# Autodesk Inventor assembly: Speaker
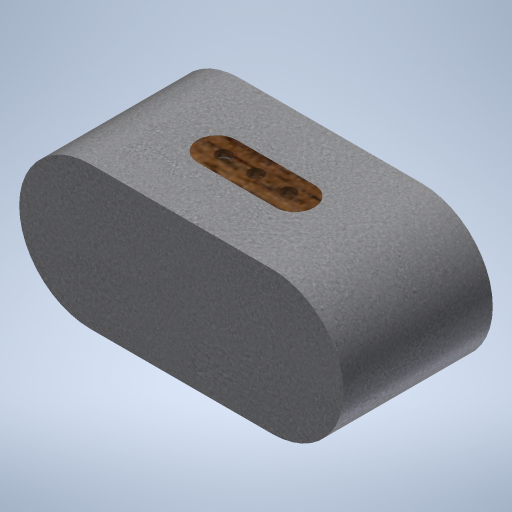
[picture p0: Inventor's stored thumbnail of the model, 512x512]
Saved by Autodesk Inventor 2023 (Build 270158000, 158)
## iProperties
Created: 2017-10-06
Part Number: Speaker
Document SubType Name: Assembly
Designer: Jared
Author: Jared
## Documents named in this file (4)
- C:\Users\Jared\Documents\GrabCAD\concrete-bluetooth-speaker\assembly.iam
- C:\Users\Jared\Documents\GrabCAD\concrete-bluetooth-speaker\concrete_case.ipt
- C:\Users\Jared\Documents\GrabCAD\concrete-bluetooth-speaker\front_panel.ipt
- C:\Users\Jared\Documents\GrabCAD\concrete-bluetooth-speaker\top_panel.ipt
## Components (3 placed, 3 different names)
1. concrete_case:1 — Mate:1, Mate:2, Mate:3, Mate:4, Flush:1, Flush:2
2. front_panel:1 — Mate:1, Mate:2, Flush:1
3. top_panel:1 — Mate:3, Mate:4, Flush:2
## Relationships (6: Mate 4, Flush 2)
- Mate:1: concrete_case:1 ↔ front_panel:1
- Mate:2: concrete_case:1 ↔ front_panel:1
- Mate:3: concrete_case:1 ↔ top_panel:1
- Mate:4: concrete_case:1 ↔ top_panel:1
- Flush:1 (12.7 mm): concrete_case:1 ↔ front_panel:1
- Flush:2: concrete_case:1 ↔ top_panel:1
